# Autodesk Inventor assembly: Piston Flag assy
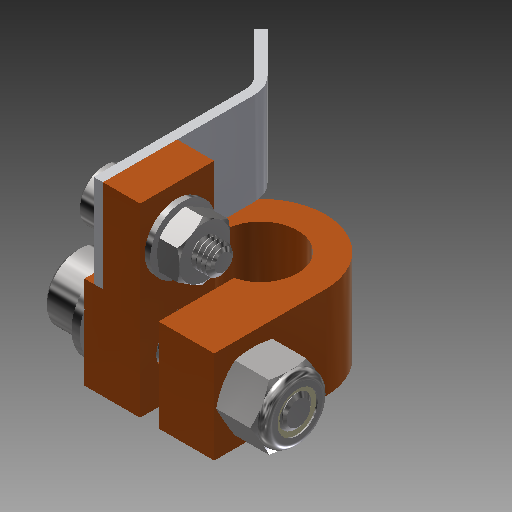
[picture p0: Inventor's stored thumbnail of the model, 512x512]
Saved by Autodesk Inventor 2018 (Build 220112000, 112)
## iProperties
Created: 2017-09-27
Part Number: Piston Flag assy
Document SubType Name: Assembly
Designer: Gabriel Smolnycki
Author: Gabriel Smolnycki
## Documents named in this file (9)
- E:\planb\mechanics\V1INV\Subassemblies\Piston Flag assy.iam
- E:\planb\mechanics\V1INV\Piston\Piston Flag Holder.ipt
- E:\planb\mechanics\V1INV\Piston\Piston Flag.ipt
- E:\planb\mechanics\V1INV\Hardware\M3 SS Washer.ipt
- E:\planb\mechanics\V1INV\Hardware\M3x10 SS SHCS.ipt
- E:\planb\mechanics\V1INV\Hardware\M3 SS Nut.ipt
- E:\planb\mechanics\V1INV\Hardware\M4 SS Washer.ipt
- E:\planb\mechanics\V1INV\Hardware\M4x20 SS SHCS.ipt
- E:\planb\mechanics\V1INV\Hardware\M4 SS Locknut.ipt
## Components (8 placed, 8 different names)
1. Piston Flag Holder:1 — Insert:1, Flush:1, Insert:3, Insert:5, Insert:7
2. Piston Flag:1 — Insert:1, Flush:1, Insert:2
3. M3 SS Washer:1 — Insert:3, Insert:4
4. M3x10 SS SHCS:1 — Insert:2
5. M3 SS Nut:1 — Insert:4
6. M4 SS Washer:1 — Insert:5, Insert:6
7. M4x20 SS SHCS:1 — Insert:6
8. M4 SS Locknut:1 — Insert:7
## Relationships (8: Insert 7, Flush 1)
- Insert:1: Piston Flag Holder:1 ↔ Piston Flag:1
- Flush:1: Piston Flag Holder:1 ↔ Piston Flag:1
- Insert:2: Piston Flag:1 ↔ M3x10 SS SHCS:1
- Insert:3: Piston Flag Holder:1 ↔ M3 SS Washer:1
- Insert:4: M3 SS Washer:1 ↔ M3 SS Nut:1
- Insert:5: Piston Flag Holder:1 ↔ M4 SS Washer:1
- Insert:6: M4 SS Washer:1 ↔ M4x20 SS SHCS:1
- Insert:7: Piston Flag Holder:1 ↔ M4 SS Locknut:1
